# Autodesk Inventor assembly: BASE_ASSEMBLY
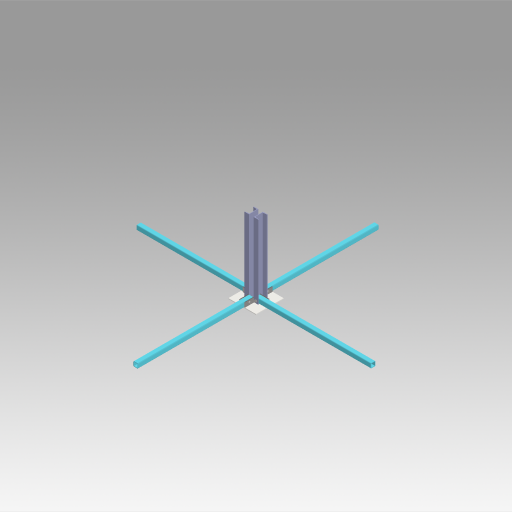
[picture p0: Inventor's stored thumbnail of the model, 512x512]
Saved by Autodesk Inventor 2023 (Build 270158000, 158)
## iProperties
Created: 2025-04-10
Part Number: BASE_ASSEMBLY
Document SubType Name: Assembly
Designer: NELLY NDUNG'U
Author: NELLY NDUNG'U
## Documents named in this file (6)
- N:\NAKUJA\CAD FILES\AIRFRAME\LP003\BASE_ASSEMBLY.iam
- N:\NAKUJA\CAD FILES\AIRFRAME\LP003\BASE PLATE.ipt
- N:\NAKUJA\CAD FILES\AIRFRAME\LP003\CHANNEL_LEG ASSEMBLY.iam
- N:\NAKUJA\CAD FILES\AIRFRAME\LP003\LEG_50.iam
- C:\Users\User\Documents\Inventor\Content Center Files\R2023\en-US\ANSI B18.2.3.5M\ANSI B18.2.3.5M - M16 x 2 x 75.ipt
- C:\Users\User\Documents\Inventor\Content Center Files\R2023\en-US\ANSI B 18.2.4.1 M(1)\ANSI B 18.2.4.1 M - M16 x 2Style 1.ipt
## Components (9 placed, 5 different names)
1. BASE PLATE:1 — Mate:1, Flush:2, Mate:2, Mate:3, Mate:4, Flush:3, Mate:5, Mate:8
2. CHANNEL_LEG ASSEMBLY:1 [sub-assembly] — Mate:1, Flush:2, Mate:2, Mate:10, Insert:3, Insert:4
3. CHANNEL_LEG ASSEMBLY:2 [sub-assembly] — Mate:3, Mate:4, Flush:3, Mate:6, Mate:7, Mate:9, Insert:1, Insert:2
4. LEG_50:1 [sub-assembly] — Mate:5, Mate:6, Mate:7
5. LEG_50:2 [sub-assembly] — Mate:8, Mate:9, Mate:10
6. Hex Bolt - Metric M16 x 2 x 75:1 — Insert:1
7. Hex Bolt - Metric M16 x 2 x 75:2 — Insert:2
8. Hex Nut Metric M16 x 2:1 — Insert:3
9. Hex Nut Metric M16 x 2:2 — Insert:4
## Relationships (16: Mate 10, Insert 4, Flush 2)
- Mate:1 (-125 mm): BASE PLATE:1 ↔ CHANNEL_LEG ASSEMBLY:1
- Flush:2 (100 mm): BASE PLATE:1 ↔ CHANNEL_LEG ASSEMBLY:1
- Mate:2: BASE PLATE:1 ↔ CHANNEL_LEG ASSEMBLY:1
- Mate:3 (-125 mm): BASE PLATE:1 ↔ CHANNEL_LEG ASSEMBLY:2
- Mate:4: BASE PLATE:1 ↔ CHANNEL_LEG ASSEMBLY:2
- Flush:3 (100 mm): BASE PLATE:1 ↔ CHANNEL_LEG ASSEMBLY:2
- Mate:5: BASE PLATE:1 ↔ LEG_50:1
- Mate:6: CHANNEL_LEG ASSEMBLY:2 ↔ LEG_50:1
- Mate:7 (5 mm): CHANNEL_LEG ASSEMBLY:2 ↔ LEG_50:1
- Mate:8: BASE PLATE:1 ↔ LEG_50:2
- Mate:9: CHANNEL_LEG ASSEMBLY:2 ↔ LEG_50:2
- Mate:10 (5 mm): CHANNEL_LEG ASSEMBLY:1 ↔ LEG_50:2
- Insert:1: CHANNEL_LEG ASSEMBLY:2 ↔ Hex Bolt - Metric M16 x 2 x 75:1
- Insert:2: CHANNEL_LEG ASSEMBLY:2 ↔ Hex Bolt - Metric M16 x 2 x 75:2
- Insert:3: CHANNEL_LEG ASSEMBLY:1 ↔ Hex Nut Metric M16 x 2:1
- Insert:4: CHANNEL_LEG ASSEMBLY:1 ↔ Hex Nut Metric M16 x 2:2
